# Autodesk Inventor assembly: ASY MSC 300.2 LEFT BOARD
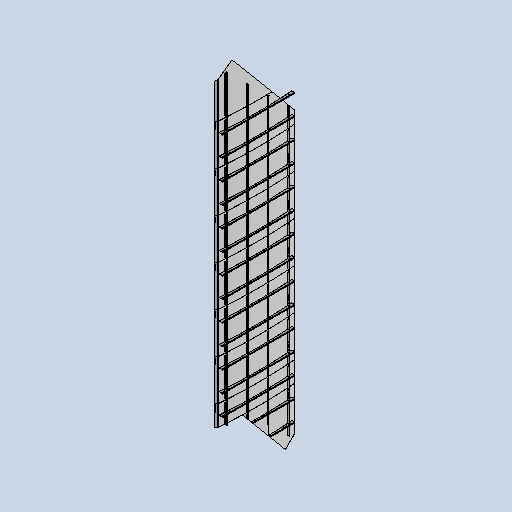
[picture p0: Inventor's stored thumbnail of the model, 512x512]
Saved by Autodesk Inventor 2025.1 (Build 291241020, 241B)
## iProperties
Created: 2024-07-21
Part Number: ASY MSC 300.2 LEFT BOARD
Document SubType Name: Assembly
Designer: pokla
Stock Number: ASY МОО 300.2 левый борт
Author: pokla
## Documents named in this file (18)
- C:\Users\user\YandexDisk-badmisterfox\домашниий пк\Inventor\Manturovo\Manturovo_Se-clar\ASY MSC 300.2 LEFT BOARD.iam
- C:\Users\user\YandexDisk-badmisterfox\домашниий пк\Inventor\Manturovo\Manturovo_Se-clar\MSC 305 RIB BOARD.ipt
- C:\Users\user\YandexDisk-badmisterfox\домашниий пк\Inventor\Manturovo\Manturovo_Se-clar\MSC 302 SHEET BOARD MAIN.ipt
- C:\Users\user\YandexDisk-badmisterfox\домашниий пк\Inventor\Manturovo\Manturovo_Se-clar\MSC 301 SHEET LEFT-RIGHT BOARD HIP.ipt
- C:\Users\user\YandexDisk-badmisterfox\домашниий пк\Inventor\Manturovo\Manturovo_Se-clar\MSC 310 SHEET LEFT BOARD WITHERS.ipt
- C:\Users\user\YandexDisk-badmisterfox\домашниий пк\Inventor\Manturovo\Manturovo_Se-clar\MSC 311 SHEET LEFT BOARD FACE.ipt
- C:\Users\user\YandexDisk-badmisterfox\домашниий пк\Inventor\Manturovo\Manturovo_Se-clar\MSC 306 stringer BOARD  #.ipt
- C:\Users\user\YandexDisk-badmisterfox\домашниий пк\Inventor\Manturovo\Manturovo_Se-clar\MSC 307 stringer BOARD  ##.ipt
- C:\Users\user\YandexDisk-badmisterfox\домашниий пк\Inventor\Manturovo\Manturovo_Se-clar\MSC 308 stringer BOARD  ###.ipt
- C:\Users\user\YandexDisk-badmisterfox\домашниий пк\Inventor\Manturovo\Manturovo_Se-clar\MSC 309 stringer BOARD  ####.ipt
- C:\Users\user\YandexDisk-badmisterfox\домашниий пк\Inventor\Manturovo\Manturovo_Se-clar\MSC 313 sheet left board hip.ipt
- C:\Users\user\YandexDisk-badmisterfox\домашниий пк\Inventor\Manturovo\Manturovo_Se-clar\MSC 316 stringer board #.ipt
- C:\Users\user\YandexDisk-badmisterfox\домашниий пк\Inventor\Manturovo\Manturovo_Se-clar\MSC 317 stringer board ##.ipt
- C:\Users\user\YandexDisk-badmisterfox\домашниий пк\Inventor\Manturovo\Manturovo_Se-clar\MSC 318 stringer BOARD  ####.ipt
- C:\Users\user\YandexDisk-badmisterfox\домашниий пк\Inventor\Manturovo\Manturovo_Se-clar\MSC 315 RIB HIP.ipt
- C:\Users\user\YandexDisk-badmisterfox\домашниий пк\Inventor\Manturovo\Manturovo_Se-clar\MSC 314 RIB HIP.ipt
- C:\Users\user\YandexDisk-badmisterfox\домашниий пк\Inventor\Manturovo\Manturovo_Se-clar\MSC 319 stringer BOARD  ###.ipt
- C:\Users\user\YandexDisk-badmisterfox\домашниий пк\Inventor\Manturovo\Manturovo_Se-clar\MSC 320 stringer board ##.ipt
## Components (55 placed, 18 different names)
1. MSC 301 SHEET LEFT-RIGHT BOARD HIP.ipt:1 — Mate:2, Rigid:20, Flush:5, Flush:6, Flush:7, Mate:3, Rigid:51
2. MSC 302 SHEET BOARD MAIN.ipt:1 — Rigid:20, Rigid:21, Flush:8, Tangent:1
3. MSC 302 SHEET BOARD MAIN.ipt:2 — Rigid:21, Rigid:22
4. MSC 302 SHEET BOARD MAIN.ipt:3 — Rigid:22, Rigid:23
5. MSC 302 SHEET BOARD MAIN.ipt:4 — Rigid:23, Rigid:24
6. MSC 302 SHEET BOARD MAIN.ipt:5 — Rigid:24, Rigid:25
7. MSC 310 SHEET LEFT BOARD WITHERS.ipt:1 — Rigid:25, Rigid:26
8. MSC 311 SHEET LEFT BOARD FACE.ipt:1 — Rigid:26
9. MSC 305 RIB BOARD.ipt:1
10. MSC 306 stringer BOARD  #.ipt:1 — Rigid:44
11. MSC 307 stringer BOARD  ##.ipt:1 — Rigid:40, Flush:8, Rigid:45
12. MSC 308 stringer BOARD  ###.ipt:2 — Rigid:41
13. MSC 309 stringer BOARD  ####.ipt:2 — Rigid:42
14. MSC 305 RIB BOARD.ipt:2
15. MSC 308 stringer BOARD  ###.ipt:1 — Rigid:49
16. MSC 309 stringer BOARD  ####.ipt:1 — Rigid:42, Rigid:46
17. MSC 305 RIB BOARD.ipt:3 — Tangent:1, Mate:3
18. MSC 313 sheet left board hip.ipt:1 — Rigid:51
19. MSC 316 stringer board #.ipt:1 — Rigid:44, Rigid:47, Rigid:48
20. MSC 317 stringer board ##.ipt:1 — Rigid:45, Rigid:50
21. MSC 318 stringer BOARD  ####.ipt:1 — Rigid:46
22. MSC 315 RIB HIP.ipt:1 — Rigid:48
23. MSC 314 RIB HIP.ipt:1 — Rigid:47
24. MSC 319 stringer BOARD  ###.ipt:1 — Rigid:49
25. MSC 320 stringer board ##.ipt:1 — Rigid:50
26. MSC 305 RIB BOARD.ipt:4
27. MSC 305 RIB BOARD.ipt:5
28. MSC 305 RIB BOARD.ipt:6
29. MSC 305 RIB BOARD.ipt:7
30. MSC 305 RIB BOARD.ipt:8
31. MSC 305 RIB BOARD.ipt:9
32. MSC 305 RIB BOARD.ipt:10
33. MSC 305 RIB BOARD.ipt:11
34. MSC 305 RIB BOARD.ipt:12
35. MSC 305 RIB BOARD:13
36. MSC 306 stringer BOARD  #.ipt:2
37. MSC 307 stringer BOARD  ##.ipt:2 — Rigid:40
38. MSC 308 stringer BOARD  ###.ipt:3 — Rigid:41
39. MSC 309 stringer BOARD  ####.ipt:3
40. MSC 306 stringer BOARD  #.ipt:3
41. MSC 307 stringer BOARD  ##.ipt:3
42. MSC 308 stringer BOARD  ###.ipt:4
43. MSC 309 stringer BOARD  ####.ipt:4
44. MSC 306 stringer BOARD  #.ipt:4
45. MSC 307 stringer BOARD  ##.ipt:4
46. MSC 308 stringer BOARD  ###.ipt:5
47. MSC 309 stringer BOARD  ####.ipt:5
48. MSC 306 stringer BOARD  #.ipt:5
49. MSC 307 stringer BOARD  ##.ipt:5
50. MSC 308 stringer BOARD  ###.ipt:6
51. MSC 309 stringer BOARD  ####.ipt:6
52. MSC 306 stringer BOARD  #.ipt:6
53. MSC 307 stringer BOARD  ##.ipt:6
54. MSC 308 stringer BOARD  ###.ipt:7
55. MSC 309 stringer BOARD  ####.ipt:7
## Component patterns: (10 elements, first: MSC 305 RIB BOARD.ipt:4), (5 elements, first: MSC 306 stringer BOARD  #.ipt:2 + MSC 307 stringer BOARD  ##.ipt:2 + MSC 308 stringer BOARD  ###.ipt:3 + MSC 309 stringer BOARD  ####.ipt:3)
## Relationships (35: WeldJoint 28, Flush 4, Mate 2, Tangent 1)
- Mate:2: MSC 301 SHEET LEFT-RIGHT BOARD HIP.ipt:1
- Rigid:20 [WeldJoint]: MSC 301 SHEET LEFT-RIGHT BOARD HIP.ipt:1 ↔ MSC 302 SHEET BOARD MAIN.ipt:1
- Rigid:21 [WeldJoint]: MSC 302 SHEET BOARD MAIN.ipt:1 ↔ MSC 302 SHEET BOARD MAIN.ipt:2
- Rigid:22 [WeldJoint]: MSC 302 SHEET BOARD MAIN.ipt:2 ↔ MSC 302 SHEET BOARD MAIN.ipt:3
- Rigid:23 [WeldJoint]: MSC 302 SHEET BOARD MAIN.ipt:3 ↔ MSC 302 SHEET BOARD MAIN.ipt:4
- Rigid:24 [WeldJoint]: MSC 302 SHEET BOARD MAIN.ipt:4 ↔ MSC 302 SHEET BOARD MAIN.ipt:5
- Rigid:25 [WeldJoint]: MSC 302 SHEET BOARD MAIN.ipt:5 ↔ MSC 310 SHEET LEFT BOARD WITHERS.ipt:1
- Flush:5: MSC 301 SHEET LEFT-RIGHT BOARD HIP.ipt:1
- Flush:6: MSC 301 SHEET LEFT-RIGHT BOARD HIP.ipt:1
- Flush:7: MSC 301 SHEET LEFT-RIGHT BOARD HIP.ipt:1
- Rigid:26 [WeldJoint]: MSC 310 SHEET LEFT BOARD WITHERS.ipt:1 ↔ MSC 311 SHEET LEFT BOARD FACE.ipt:1
- [WeldJoint]: MSC 306 stringer BOARD  #.ipt:1 ↔ MSC 306 stringer BOARD  #.ipt:2
- [WeldJoint]: MSC 308 stringer BOARD  ###.ipt:2 ↔ MSC 308 stringer BOARD  ###.ipt:1
- [WeldJoint]: MSC 309 stringer BOARD  ####.ipt:2 ↔ MSC 309 stringer BOARD  ####.ipt:3
- [WeldJoint] (2 mm): MSC 305 RIB BOARD.ipt:1 ↔ MSC 306 stringer BOARD  #.ipt:2
- [WeldJoint] (2 mm): MSC 306 stringer BOARD  #.ipt:1 ↔ MSC 305 RIB BOARD.ipt:2
- [WeldJoint] (2 mm): MSC 306 stringer BOARD  #.ipt:1 ↔ MSC 305 RIB BOARD.ipt:3
- [WeldJoint] (2 mm): MSC 305 RIB BOARD.ipt:1 ↔ MSC 309 stringer BOARD  ####.ipt:1
- [WeldJoint] (2 mm): MSC 305 RIB BOARD.ipt:1 ↔ MSC 307 stringer BOARD  ##.ipt:1
- [WeldJoint] (2 mm): MSC 305 RIB BOARD.ipt:1 ↔ MSC 308 stringer BOARD  ###.ipt:2
- [WeldJoint] (2 mm): MSC 305 RIB BOARD.ipt:4 ↔ MSC 306 stringer BOARD  #.ipt:2
- Rigid:40 [WeldJoint]: MSC 307 stringer BOARD  ##.ipt:1 ↔ MSC 307 stringer BOARD  ##.ipt:2
- Rigid:41 [WeldJoint]: MSC 308 stringer BOARD  ###.ipt:2 ↔ MSC 308 stringer BOARD  ###.ipt:3
- Rigid:42 [WeldJoint]: MSC 309 stringer BOARD  ####.ipt:2 ↔ MSC 309 stringer BOARD  ####.ipt:1
- Flush:8 (-2 mm): MSC 302 SHEET BOARD MAIN.ipt:1 ↔ MSC 307 stringer BOARD  ##.ipt:1
- Tangent:1: MSC 302 SHEET BOARD MAIN.ipt:1 ↔ MSC 305 RIB BOARD.ipt:3
- Mate:3 (-75 mm): MSC 301 SHEET LEFT-RIGHT BOARD HIP.ipt:1 ↔ MSC 305 RIB BOARD.ipt:3
- Rigid:44 [WeldJoint]: MSC 306 stringer BOARD  #.ipt:1 ↔ MSC 316 stringer board #.ipt:1
- Rigid:45 [WeldJoint]: MSC 307 stringer BOARD  ##.ipt:1 ↔ MSC 317 stringer board ##.ipt:1
- Rigid:46 [WeldJoint]: MSC 309 stringer BOARD  ####.ipt:1 ↔ MSC 318 stringer BOARD  ####.ipt:1
- Rigid:47 [WeldJoint] (2 mm): MSC 316 stringer board #.ipt:1 ↔ MSC 314 RIB HIP.ipt:1
- Rigid:48 [WeldJoint] (2 mm): MSC 316 stringer board #.ipt:1 ↔ MSC 315 RIB HIP.ipt:1
- Rigid:49 [WeldJoint]: MSC 308 stringer BOARD  ###.ipt:1 ↔ MSC 319 stringer BOARD  ###.ipt:1
- Rigid:50 [WeldJoint]: MSC 317 stringer board ##.ipt:1 ↔ MSC 320 stringer board ##.ipt:1
- Rigid:51 [WeldJoint]: MSC 301 SHEET LEFT-RIGHT BOARD HIP.ipt:1 ↔ MSC 313 sheet left board hip.ipt:1
